# Autodesk Inventor assembly: one-of-each
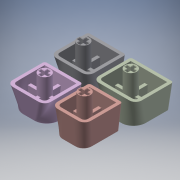
[picture p0: Inventor's stored thumbnail of the model, 180x180]
Saved by Autodesk Inventor 2016 (Build 200138000, 138)
## iProperties
Created: 2016-12-15
Part Number: one-of-each
Document SubType Name: Assembly
Designer: Cemra JC
Author: Cemra JC
## Documents named in this file (6)
- J:\The Files\The Software Files\Projects\stenotoppers\cherrymx\print-assemblies\one-of-each.iam
- J:\The Files\The Software Files\Projects\stenotoppers\cherrymx\stenotoppers\standard_cmx.ipt
- J:\The Files\The Software Files\Projects\stenotoppers\cherrymx\stenotoppers.ipt
- J:\The Files\The Software Files\Projects\stenotoppers\cherrymx\stenotoppers\smaller_cmx.ipt
- J:\The Files\The Software Files\Projects\stenotoppers\cherrymx\stenotoppers\larger_cmx.ipt
- J:\The Files\The Software Files\Projects\stenotoppers\cherrymx\stenotoppers\thumb_cmx.ipt
## Components (4 placed, 4 different names)
1. standard_cmx:1 — Flush:2
2. smaller_cmx:2 — Flush:3
3. larger_cmx:3 — Flush:1
4. thumb_cmx:4 — Flush:1, Flush:2, Flush:3
## Relationships (3: Flush 3)
- Flush:1: larger_cmx:3 ↔ thumb_cmx:4
- Flush:2: standard_cmx:1 ↔ thumb_cmx:4
- Flush:3: smaller_cmx:2 ↔ thumb_cmx:4
